# Autodesk Inventor assembly: ASY PNS 1752 FDS way 2_1600
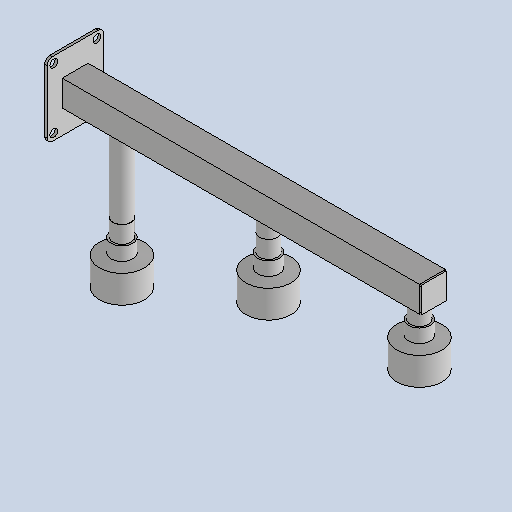
[picture p0: Inventor's stored thumbnail of the model, 512x512]
Saved by Autodesk Inventor 2025.1 (Build 291241020, 241B)
## iProperties
Created: 2025-07-02
Part Number: ASY PNS 1752 FDS way 2_1600
Document SubType Name: Assembly
Designer: admin
Author: user
## Documents named in this file (8)
- C:\Users\user\YandexDisk-badmisterfox\home pc\Inventor\PNS2-Panaevsk\Filter D1000\filter-distribution-system 1000\ASY PNS 1752 FDS way 2_1600.iam
- C:\Users\user\YandexDisk-badmisterfox\home pc\Inventor\PNS2-Panaevsk\Filter D1000\filter-distribution-system 1000\PNS 1752 FDS 1200 way tube 2_1600.ipt
- C:\Users\user\YandexDisk-badmisterfox\home pc\Inventor\PNS2-Panaevsk\Filter D1000\filter-distribution-system 1000\PNS dummy filter element_1600.ipt
- C:\Users\user\YandexDisk-badmisterfox\home pc\Inventor\PNS2-Panaevsk\Filter D1000\filter-distribution-system 1000\PNS dummy pipe nippel_1600.ipt
- C:\Users\user\YandexDisk-badmisterfox\home pc\Inventor\PNS2-Panaevsk\Filter D1000\filter-distribution-system 1000\PNS 1756 FDS 1200 way tube 6_1600.ipt
- C:\Users\user\YandexDisk-badmisterfox\home pc\Inventor\PNS2-Panaevsk\Filter D1000\filter-distribution-system 1000\PNS 1757 FDS 1200 way tube 7_1600.ipt
- C:\Users\user\YandexDisk-badmisterfox\home pc\Inventor\PNS2-Panaevsk\Filter D1000\filter-distribution-system 1000\PNS 760 FDS 1200 FLANGE 3_1600.ipt
- C:\Users\user\YandexDisk-badmisterfox\home pc\Inventor\PNS2-Panaevsk\Filter D1000\filter-distribution-system 1000\PNS 766 FDS 1200 CUP 1_1600.ipt
## Components (11 placed, 7 different names)
1. PNS 1752 FDS 1200 way tube 2_1600:1 — Rigid:2, Rigid:5, Rigid:8, Rigid:9, Rigid:10
2. PNS dummy filter element_1600:1 — Rigid:1
3. PNS dummy pipe nippel_1600:1 — Rigid:2, Rigid:1
4. PNS 1756 FDS 1200 way tube 6_1600:1 — Rigid:5, Rigid:4
5. PNS dummy filter element_1600:2 — Rigid:3
6. PNS dummy pipe nippel_1600:2 — Rigid:4, Rigid:3
7. PNS 1757 FDS 1200 way tube 7_1600:1 — Rigid:8, Rigid:7
8. PNS dummy filter element_1600:3 — Rigid:6
9. PNS dummy pipe nippel_1600:3 — Rigid:7, Rigid:6
10. PNS 760 FDS 1200 FLANGE 3_1600:1 — Rigid:9
11. PNS 766 FDS 1200 CUP 1_1600:1 — Rigid:10
## Relationships (10: WeldJoint 10)
- Rigid:2 [WeldJoint]: PNS 1752 FDS 1200 way tube 2_1600:1 ↔ PNS dummy pipe nippel_1600:1
- Rigid:1 [WeldJoint]: PNS dummy filter element_1600:1 ↔ PNS dummy pipe nippel_1600:1
- Rigid:5 [WeldJoint]: PNS 1752 FDS 1200 way tube 2_1600:1 ↔ PNS 1756 FDS 1200 way tube 6_1600:1
- Rigid:4 [WeldJoint]: PNS 1756 FDS 1200 way tube 6_1600:1 ↔ PNS dummy pipe nippel_1600:2
- Rigid:3 [WeldJoint]: PNS dummy filter element_1600:2 ↔ PNS dummy pipe nippel_1600:2
- Rigid:8 [WeldJoint]: PNS 1752 FDS 1200 way tube 2_1600:1 ↔ PNS 1757 FDS 1200 way tube 7_1600:1
- Rigid:7 [WeldJoint]: PNS 1757 FDS 1200 way tube 7_1600:1 ↔ PNS dummy pipe nippel_1600:3
- Rigid:6 [WeldJoint]: PNS dummy filter element_1600:3 ↔ PNS dummy pipe nippel_1600:3
- Rigid:9 [WeldJoint] (-3 mm): PNS 1752 FDS 1200 way tube 2_1600:1 ↔ PNS 760 FDS 1200 FLANGE 3_1600:1
- Rigid:10 [WeldJoint]: PNS 1752 FDS 1200 way tube 2_1600:1 ↔ PNS 766 FDS 1200 CUP 1_1600:1
